# Autodesk Inventor assembly: Palma_final
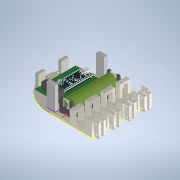
[picture p0: Inventor's stored thumbnail of the model, 180x180]
Saved by Autodesk Inventor 2020.4 (Build 244396010, 396A)
## iProperties
Created: 2021-11-22
Part Number: Palma_final
Document SubType Name: Assembly
Designer: chalo
Author: chalo
## Documents named in this file (5)
- C:\Users\chalo\OneDrive\Documents\GitHub\Interfaces-Biomedicas-2021\Gonzalo Palarea\Inventor\Ensamblaje_Final\Palma_final.iam
- C:\Users\chalo\OneDrive\Documents\GitHub\Interfaces-Biomedicas-2021\Gonzalo Palarea\Inventor\Ensamblaje_Final\ipts\Palma.ipt
- C:\Users\chalo\OneDrive\Documents\GitHub\Interfaces-Biomedicas-2021\Gonzalo Palarea\Inventor\referencias\18650.ipt
- C:\Users\chalo\OneDrive\Documents\GitHub\Interfaces-Biomedicas-2021\Gonzalo Palarea\Inventor\referencias\Battery Holder 18650_COMF_BHC-18650-1A.ipt
- C:\Users\chalo\OneDrive\Documents\GitHub\Interfaces-Biomedicas-2021\Gonzalo Palarea\Inventor\referencias\PCB_Prueba.iam
## Components (4 placed, 4 different names)
1. Palma:1
2. 18650:1
3. Battery Holder 18650_COMF_BHC-18650-1A:1 — Angle:1
4. PCB_Prueba:1 [sub-assembly] — Angle:2
## Relationships (2: Angle 2)
- Angle:1 (0 deg): Battery Holder 18650_COMF_BHC-18650-1A:1
- Angle:2 (0 deg): PCB_Prueba:1
